# Autodesk Inventor assembly: LowerFrontLink
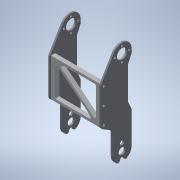
[picture p0: Inventor's stored thumbnail of the model, 180x180]
Saved by Autodesk Inventor 2020 (Build 240168000, 168)
## iProperties
Created: 2016-08-23
Part Number: LowerFrontLink
Material: 一般
Document SubType Name: Assembly
Designer: hiro
Mass: 33.5175 g
Surface Area: 182.778 cm^2
Volume: 15.549 cm^3
Density: 2.15561 g/cm^3
Author: hiro
## Documents named in this file (3)
- C:\Users\Masato\Desktop\最新版\OpenPlatform_ver3_0\下半身\リンク\LowerFrontLink.iam
- C:\Users\Masato\Desktop\最新版\OpenPlatform_ver3_0\下半身\リンク\リンク_ふくらはぎ_サブフレーム_1_1.ipt
- C:\Users\Masato\Desktop\最新版\OpenPlatform_ver3_0\下半身\リンク\リンク_メインフレーム_6_4.ipt
## Components (3 placed, 2 different names)
1. リンク_メインフレーム_6_4:1 — 挿入:7, 挿入:8, 挿入:9
2. リンク_メインフレーム_6_4:2 — 挿入:10, 挿入:11, 挿入:12
3. リンク_ふくらはぎ_サブフレーム_1_1:1 — 挿入:7, 挿入:8, 挿入:9, 挿入:10, 挿入:11, 挿入:12
## Relationships (6: Insert 6)
- 挿入:7 [Insert]: リンク_メインフレーム_6_4:1 ↔ リンク_ふくらはぎ_サブフレーム_1_1:1
- 挿入:8 [Insert]: リンク_メインフレーム_6_4:1 ↔ リンク_ふくらはぎ_サブフレーム_1_1:1
- 挿入:9 [Insert]: リンク_メインフレーム_6_4:1 ↔ リンク_ふくらはぎ_サブフレーム_1_1:1
- 挿入:10 [Insert]: リンク_メインフレーム_6_4:2 ↔ リンク_ふくらはぎ_サブフレーム_1_1:1
- 挿入:11 [Insert]: リンク_メインフレーム_6_4:2 ↔ リンク_ふくらはぎ_サブフレーム_1_1:1
- 挿入:12 [Insert]: リンク_メインフレーム_6_4:2 ↔ リンク_ふくらはぎ_サブフレーム_1_1:1
